# Autodesk Inventor assembly: test_assy
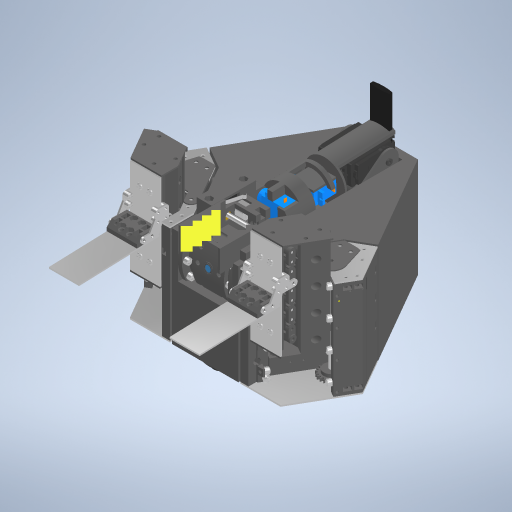
[picture p0: Inventor's stored thumbnail of the model, 512x512]
Saved by Autodesk Inventor 2024.1 (Build 281209000, 209)
## iProperties
Created: 2025-01-17
Part Number: test_assy
Document SubType Name: Assembly
Designer: hibik
Author: hibik
## Documents named in this file (9)
- C:\Users\hibik\Documents\Robomech\RESCUE\ORCA\hard\test_assy.iam
- C:\Users\hibik\Documents\Robomech\RESCUE\ORCA\hard\camera\cam_set.iam
- C:\Users\hibik\Documents\Robomech\RESCUE\ORCA\hard\omni_wheel\wheel_set.iam
- C:\Users\hibik\Documents\Robomech\RESCUE\ORCA\hard\fork\right\Assy_fork_right.iam
- C:\Users\hibik\Documents\Robomech\RESCUE\ORCA\hard\fork\Assy_fork_left_test.iam
- C:\Users\hibik\Documents\Robomech\RESCUE\ORCA\hard\std_parts\Buffalo_Wl-U2-433DHP.ipt
- C:\Users\hibik\Documents\Robomech\RESCUE\ORCA\hard\arm\arm_test.iam
- C:\Users\hibik\Documents\Robomech\RESCUE\ORCA\hard\arm\arm_base.ipt
- C:\Users\hibik\Documents\Robomech\RESCUE\ORCA\hard\cover.ipt
## Components (10 placed, 8 different names)
1. cam_set:1 [sub-assembly] — フラッシュ:4, 角度:8
2. wheel_set:1 [sub-assembly] — 角度:3, 角度:4, 角度:5, メイト:3, フラッシュ:1
3. wheel_set:2 [sub-assembly] — 角度:2, 角度:3, メイト:2, フラッシュ:2
4. wheel_set:3 [sub-assembly] — 角度:1, 角度:4, メイト:1, フラッシュ:3
5. Assy_fork_right:1 [sub-assembly]
6. Assy_fork_left_test:1 [sub-assembly]
7. Buffalo_Wl-U2-433DHP:1
8. arm_test:1 [sub-assembly] — 挿入:1
9. arm_base:1 — 角度:9, フラッシュ:6, フラッシュ:7, メイト:6, 挿入:1
10. cover:1 — フラッシュ:8, フラッシュ:9, フラッシュ:10
## Relationships (26: Flush 10, Angle 9, Mate 6, Insert 1)
- 角度:1 [Angle] (0 deg): wheel_set:3
- 角度:2 [Angle] (0 deg): wheel_set:2
- 角度:3 [Angle] (-120 deg): wheel_set:1 ↔ wheel_set:2
- 角度:4 [Angle] (-120 deg): wheel_set:1 ↔ wheel_set:3
- 角度:5 [Angle] (0 deg): wheel_set:1
- メイト:1 [Mate]: wheel_set:3
- メイト:2 [Mate]: wheel_set:2
- メイト:3 [Mate]: wheel_set:1
- メイト:4 [Mate]
- 角度:6 [Angle] (60 deg)
- メイト:5 [Mate]
- 角度:7 [Angle] (-60 deg)
- フラッシュ:1 [Flush] (-37.5 mm): wheel_set:1
- フラッシュ:2 [Flush] (-37.5 mm): wheel_set:2
- フラッシュ:3 [Flush] (-37.5 mm): wheel_set:3
- フラッシュ:4 [Flush] (-26.9 mm): cam_set:1
- フラッシュ:5 [Flush] (100 mm)
- 角度:8 [Angle] (0 deg): cam_set:1
- 角度:9 [Angle] (180 deg): arm_base:1
- フラッシュ:6 [Flush] (-20 mm): arm_base:1
- フラッシュ:7 [Flush] (83 mm): arm_base:1
- メイト:6 [Mate] (75 mm): arm_base:1
- 挿入:1 [Insert]: arm_test:1 ↔ arm_base:1
- フラッシュ:8 [Flush]: cover:1
- フラッシュ:9 [Flush]: cover:1
- フラッシュ:10 [Flush]: cover:1
